# Autodesk Inventor assembly: tableStand
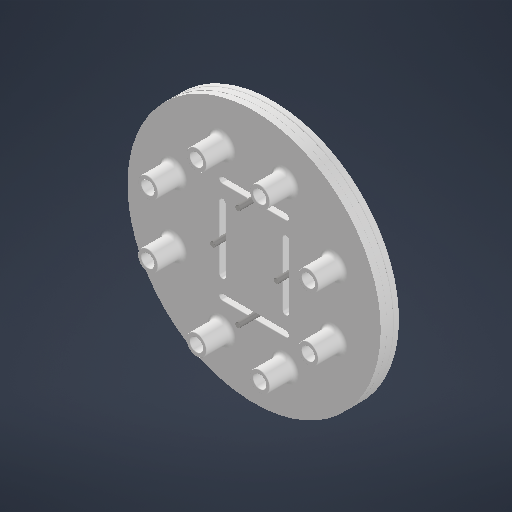
[picture p0: Inventor's stored thumbnail of the model, 512x512]
Saved by Autodesk Inventor 2026.3 (Build 303398000, 398)
## iProperties
Created: 2026-06-26
Part Number: tableStand
Document SubType Name: Assembly
Designer: frede
Author: frede
## Documents named in this file (5)
- E:\Git\AppliedAutomationProject\CAD\feeder\tableStand.iam
- E:\Git\AppliedAutomationProject\CAD\feeder\tableStandBottom.ipt
- D:\OneDrive\Dokumenter\Inventor\Content Center Files\R2026\en-US\BS EN ISO 4017\BS EN ISO 4017 - M4 x 20BS EN.ipt
- E:\Git\AppliedAutomationProject\CAD\feeder\TableStandMiddle.ipt
- E:\Git\AppliedAutomationProject\CAD\feeder\tableStandTop.ipt
## Components (7 placed, 4 different names)
1. tableStandBottom:1 — Mate:1, Mate:2, Mate:3, Mate:4, Angle:1, Angle:2, Flush:1
2. BS EN ISO 4017 - Metric M4 x 20:1 — Mate:1, Mate:2, Angle:1
3. BS EN ISO 4017 - Metric M4 x 20:2 — Mate:3, Mate:4, Angle:2
4. TableStandMiddle:1 — Flush:1, Insert:1, Insert:2, Flush:2
5. BS EN ISO 4017 - Metric M4 x 20:3 — Insert:1
6. BS EN ISO 4017 - Metric M4 x 20:4 — Insert:2
7. tableStandTop:1 — Flush:2
## Relationships (10: Mate 4, Angle 2, Flush 2, Insert 2)
- Mate:1: tableStandBottom:1 ↔ BS EN ISO 4017 - Metric M4 x 20:1
- Mate:2: tableStandBottom:1 ↔ BS EN ISO 4017 - Metric M4 x 20:1
- Mate:3: tableStandBottom:1 ↔ BS EN ISO 4017 - Metric M4 x 20:2
- Mate:4: tableStandBottom:1 ↔ BS EN ISO 4017 - Metric M4 x 20:2
- Angle:1 (0 deg): tableStandBottom:1 ↔ BS EN ISO 4017 - Metric M4 x 20:1
- Angle:2 (0 deg): tableStandBottom:1 ↔ BS EN ISO 4017 - Metric M4 x 20:2
- Flush:1: tableStandBottom:1 ↔ TableStandMiddle:1
- Insert:1: TableStandMiddle:1 ↔ BS EN ISO 4017 - Metric M4 x 20:3
- Insert:2: TableStandMiddle:1 ↔ BS EN ISO 4017 - Metric M4 x 20:4
- Flush:2: TableStandMiddle:1 ↔ tableStandTop:1
